# Autodesk Inventor assembly: Left Door
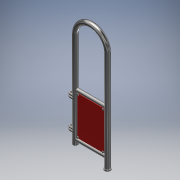
[picture p0: Inventor's stored thumbnail of the model, 180x180]
Saved by Autodesk Inventor 2018 (Build 220112000, 112)
## iProperties
Created: 2018-02-10
Part Number: Left Door
Document SubType Name: Assembly
Designer: Joey
Author: Joey
## Documents named in this file (5)
- C:\Users\Joey\Desktop\School\CADD 2\Ferris Wheel\Left Door.iam
- C:\Users\Joey\Desktop\School\CADD 2\Ferris Wheel\Door Frame.ipt
- C:\Users\Joey\Desktop\School\CADD 2\Ferris Wheel\Door Plate Nut.ipt
- C:\Users\Joey\Desktop\School\CADD 2\Ferris Wheel\Door Plate Screw.ipt
- C:\Users\Joey\Desktop\School\CADD 2\Ferris Wheel\Door Plate.ipt
## Components (10 placed, 4 different names)
1. Door Frame:1 — Flush:1
2. Door Plate Nut:1 — Insert:8
3. Door Plate Screw:1 — Insert:1, Insert:5
4. Door Plate Nut:2 — Insert:6
5. Door Plate Screw:2 — Insert:4, Insert:6
6. Door Plate Nut:3 — Insert:5
7. Door Plate Screw:3 — Insert:2, Insert:8
8. Door Plate Nut:4 — Insert:7
9. Door Plate Screw:4 — Insert:3, Insert:7
10. Door Plate:1 — Flush:1, Insert:1, Insert:2, Insert:3, Insert:4
## Relationships (9: Insert 8, Flush 1)
- Flush:1: Door Frame:1 ↔ Door Plate:1
- Insert:1: Door Plate Screw:1 ↔ Door Plate:1
- Insert:2: Door Plate Screw:3 ↔ Door Plate:1
- Insert:3: Door Plate Screw:4 ↔ Door Plate:1
- Insert:4: Door Plate Screw:2 ↔ Door Plate:1
- Insert:5: Door Plate Screw:1 ↔ Door Plate Nut:3
- Insert:6: Door Plate Nut:2 ↔ Door Plate Screw:2
- Insert:7: Door Plate Nut:4 ↔ Door Plate Screw:4
- Insert:8: Door Plate Nut:1 ↔ Door Plate Screw:3
